# Autodesk Inventor assembly: Plotter
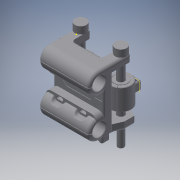
[picture p0: Inventor's stored thumbnail of the model, 180x180]
Saved by Autodesk Inventor 2018 (Build 220112000, 112)
## iProperties
Created: 2018-05-11
Part Number: Plotter
Document SubType Name: Assembly
Designer: Jasper
Author: Jasper
## Documents named in this file (8)
- D:\Jasper's Stuff\git_WSL\MEME_MACHINE\CAD\Plotter.iam
- D:\Jasper's Stuff\git_WSL\MEME_MACHINE\CAD\x-carriage-with-endstop-trigger.ipt
- D:\Jasper's Stuff\git_WSL\MEME_MACHINE\CAD\PlotterBase.ipt
- D:\Jasper's Stuff\git_WSL\MEME_MACHINE\CAD\Vitamins\PlotterScrew.ipt
- D:\Jasper's Stuff\git_WSL\MEME_MACHINE\CAD\Vitamins\lm8uu.ipt
- D:\Jasper's Stuff\git_WSL\MEME_MACHINE\CAD\PlotterPenHolder.ipt
- D:\Jasper's Stuff\git_WSL\MEME_MACHINE\CAD\PlotterPenHolderAlt.ipt
- D:\Jasper's Stuff\git_WSL\MEME_MACHINE\CAD\PlotterPenHolderAltClamp.ipt
## Components (9 placed, 7 different names)
1. x-carriage-with-endstop-trigger:1 — Flush:1, Flush:2, Flush:3
2. PlotterBase:1 — Flush:1, Flush:2, Flush:3, Mate:2, Mate:3, Mate:5, Mate:6, Angle:2, Angle:3
3. PlotterScrew:1 — Mate:1, Mate:2, Mate:3
4. PlotterScrew:2 — Mate:4, Mate:5, Mate:6
5. lm8uu:1 — Mate:4, Flush:4
6. lm8uu:2 — Mate:1, Flush:4, Flush:5, Mate:7, Mate:9, Flush:7
7. PlotterPenHolder:1 — Flush:5, Mate:7, Angle:3
8. PlotterPenHolderAlt:1 — Mate:8, Angle:1, Mate:9, Flush:7, Angle:2
9. PlotterPenHolderAltClamp:1 — Mate:8, Angle:1
## Relationships (18: Mate 9, Flush 6, Angle 3)
- Flush:1: x-carriage-with-endstop-trigger:1 ↔ PlotterBase:1
- Flush:2: x-carriage-with-endstop-trigger:1 ↔ PlotterBase:1
- Flush:3: x-carriage-with-endstop-trigger:1 ↔ PlotterBase:1
- Mate:1: PlotterScrew:1 ↔ lm8uu:2
- Mate:2: PlotterBase:1 ↔ PlotterScrew:1
- Mate:3: PlotterBase:1 ↔ PlotterScrew:1
- Mate:4: PlotterScrew:2 ↔ lm8uu:1
- Mate:5: PlotterBase:1 ↔ PlotterScrew:2
- Mate:6: PlotterBase:1 ↔ PlotterScrew:2
- Flush:4: lm8uu:1 ↔ lm8uu:2
- Flush:5: lm8uu:2 ↔ PlotterPenHolder:1
- Mate:7: lm8uu:2 ↔ PlotterPenHolder:1
- Mate:8: PlotterPenHolderAlt:1 ↔ PlotterPenHolderAltClamp:1
- Angle:1 (0 deg): PlotterPenHolderAlt:1 ↔ PlotterPenHolderAltClamp:1
- Mate:9: lm8uu:2 ↔ PlotterPenHolderAlt:1
- Flush:7: lm8uu:2 ↔ PlotterPenHolderAlt:1
- Angle:2 (180 deg): PlotterBase:1 ↔ PlotterPenHolderAlt:1
- Angle:3 (180 deg): PlotterBase:1 ↔ PlotterPenHolder:1
